# Autodesk Inventor assembly: Gear_Wheel_Assembly
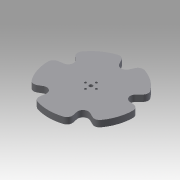
[picture p0: Inventor's stored thumbnail of the model, 180x180]
Saved by Autodesk Inventor 2016 (Build 200138000, 138)
## iProperties
Created: 2015-11-28
Part Number: Gear_Wheel_Assembly
Document SubType Name: Assembly
Designer: Delta
Author: Delta
## Documents named in this file (3)
- C:\Robotics\CAD\2015-16\custom cad parts\Gear_Wheel_Assembly.iam
- C:\Robotics\CAD\2015-16\COTSParts\Actobotics\545 parts\545548.ipt
- C:\Robotics\CAD\2015-16\custom cad parts\gear wheel.ipt
## Components (2 placed, 2 different names)
1. 545548:1 — Mate:1, Mate:2, Mate:3
2. gear wheel:1 — Mate:1, Mate:2, Mate:3
## Relationships (3: Mate 3)
- Mate:1: 545548:1 ↔ gear wheel:1
- Mate:2: 545548:1 ↔ gear wheel:1
- Mate:3: 545548:1 ↔ gear wheel:1
